# Autodesk Inventor assembly: CameraUnit_e-CAM50_CUNX
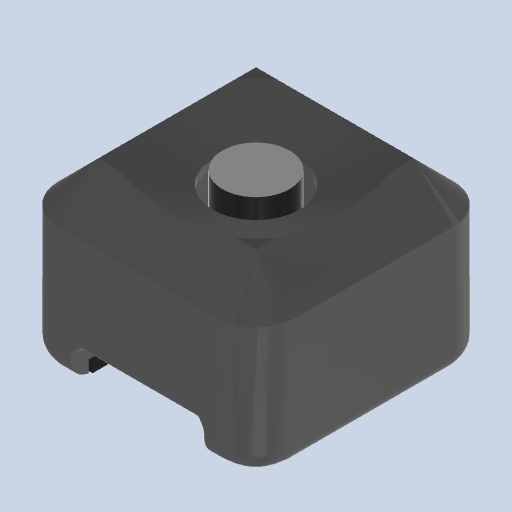
[picture p0: Inventor's stored thumbnail of the model, 512x512]
Saved by Autodesk Inventor 2022 (Build 260153000, 153)
## iProperties
Created: 2021-12-31
Part Number: CameraUnit_e-CAM50_CUNX
Document SubType Name: Assembly
Designer: Masato Kubotera
Mass: 42.9724 g
Surface Area: 234.622 cm^2
Volume: 68.7932 cm^3
Density: 0.624661 g/cm^3
Author: Masato Kubotera
## Documents named in this file (9)
- C:\Users\MasatoKubotera\Desktop\SUSTAINA-OP\UpperBody\Head\CameraUnit_e-CAM50_CUNX.iam
- C:\Users\MasatoKubotera\Desktop\SUSTAINA-OP\UpperBody\Head\Camera_root_frame_e-CAM50_CUNX.ipt
- C:\Users\MasatoKubotera\Desktop\SUSTAINA-OP\ReadyMade\InsertNut\BRM2-4.1.ipt
- C:\Users\MasatoKubotera\Desktop\SUSTAINA-OP\ReadyMade\Camera\e-CAM50_CUNX.ipt
- C:\Users\MasatoKubotera\Desktop\SUSTAINA-OP\UpperBody\Head\Camera_cover_e-CAM50_CUNX.ipt
- C:\Users\MasatoKubotera\Desktop\SUSTAINA-OP\ReadyMade\InsertNut\UD-43040.ipt
- C:\Users\MasatoKubotera\Desktop\SUSTAINA-OP\ReadyMade\Screw\M2-15.ipt
- C:\Users\MasatoKubotera\Desktop\SUSTAINA-OP\ReadyMade\Spacer\C-2006-4.ipt
- C:\Users\MasatoKubotera\Desktop\SUSTAINA-OP\ReadyMade\Spacer\C-2002.5-4.ipt
## Components (23 placed, 8 different names)
1. Camera_root_frame_e-CAM50_CUNX:1 — 挿入:1, 挿入:2, 挿入:3, 挿入:4, 挿入:17, 挿入:18, 挿入:19, 挿入:20
2. BRM2-4.1:1 — 挿入:1, 挿入:40
3. BRM2-4.1:2 — 挿入:2, 挿入:39
4. BRM2-4.1:3 — 挿入:3, 挿入:42
5. BRM2-4.1:4 — 挿入:4, 挿入:41
6. e-CAM50_CUNX:1 — 挿入:27, 挿入:28, 挿入:29, 挿入:30, 挿入:31, 挿入:32, 挿入:33, 挿入:34, 挿入:35, 挿入:36, 挿入:37, 挿入:38
7. Camera_cover_e-CAM50_CUNX:1 — 挿入:13, 挿入:14, 挿入:15, 挿入:16
8. M2-15:1 — 挿入:27
9. M2-15:2 — 挿入:28
10. M2-15:3 — 挿入:29
11. M2-15:4 — 挿入:30
12. C-2006-4:1 — 挿入:31
13. C-2006-4:2 — 挿入:32
14. C-2006-4:3 — 挿入:33
15. C-2006-4:4 — 挿入:34
16. C-2002.5-4:1 — 挿入:35, 挿入:41
17. C-2002.5-4:2 — 挿入:36, 挿入:39
18. C-2002.5-4:3 — 挿入:37, 挿入:40
19. C-2002.5-4:4 — 挿入:38, 挿入:42
20. UD-43040:1 — 挿入:13, 挿入:18
21. UD-43040:2 — 挿入:14, 挿入:17
22. UD-43040:3 — 挿入:15, 挿入:20
23. UD-43040:4 — 挿入:16, 挿入:19
## Relationships (28: Insert 28)
- 挿入:1 [Insert]: Camera_root_frame_e-CAM50_CUNX:1 ↔ BRM2-4.1:1
- 挿入:2 [Insert]: Camera_root_frame_e-CAM50_CUNX:1 ↔ BRM2-4.1:2
- 挿入:3 [Insert]: Camera_root_frame_e-CAM50_CUNX:1 ↔ BRM2-4.1:3
- 挿入:4 [Insert]: Camera_root_frame_e-CAM50_CUNX:1 ↔ BRM2-4.1:4
- 挿入:13 [Insert]: Camera_cover_e-CAM50_CUNX:1 ↔ UD-43040:1
- 挿入:14 [Insert]: Camera_cover_e-CAM50_CUNX:1 ↔ UD-43040:2
- 挿入:15 [Insert]: Camera_cover_e-CAM50_CUNX:1 ↔ UD-43040:3
- 挿入:16 [Insert]: Camera_cover_e-CAM50_CUNX:1 ↔ UD-43040:4
- 挿入:17 [Insert]: Camera_root_frame_e-CAM50_CUNX:1 ↔ UD-43040:2
- 挿入:18 [Insert]: Camera_root_frame_e-CAM50_CUNX:1 ↔ UD-43040:1
- 挿入:19 [Insert]: Camera_root_frame_e-CAM50_CUNX:1 ↔ UD-43040:4
- 挿入:20 [Insert]: Camera_root_frame_e-CAM50_CUNX:1 ↔ UD-43040:3
- 挿入:27 [Insert]: e-CAM50_CUNX:1 ↔ M2-15:1
- 挿入:28 [Insert]: e-CAM50_CUNX:1 ↔ M2-15:2
- 挿入:29 [Insert]: e-CAM50_CUNX:1 ↔ M2-15:3
- 挿入:30 [Insert]: e-CAM50_CUNX:1 ↔ M2-15:4
- 挿入:31 [Insert]: e-CAM50_CUNX:1 ↔ C-2006-4:1
- 挿入:32 [Insert]: e-CAM50_CUNX:1 ↔ C-2006-4:2
- 挿入:33 [Insert]: e-CAM50_CUNX:1 ↔ C-2006-4:3
- 挿入:34 [Insert]: e-CAM50_CUNX:1 ↔ C-2006-4:4
- 挿入:35 [Insert]: e-CAM50_CUNX:1 ↔ C-2002.5-4:1
- 挿入:36 [Insert]: e-CAM50_CUNX:1 ↔ C-2002.5-4:2
- 挿入:37 [Insert]: e-CAM50_CUNX:1 ↔ C-2002.5-4:3
- 挿入:38 [Insert]: e-CAM50_CUNX:1 ↔ C-2002.5-4:4
- 挿入:39 [Insert]: BRM2-4.1:2 ↔ C-2002.5-4:2
- 挿入:40 [Insert]: BRM2-4.1:1 ↔ C-2002.5-4:3
- 挿入:41 [Insert]: BRM2-4.1:4 ↔ C-2002.5-4:1
- 挿入:42 [Insert]: BRM2-4.1:3 ↔ C-2002.5-4:4
